# Autodesk Inventor assembly: ASY MSC 800 gills
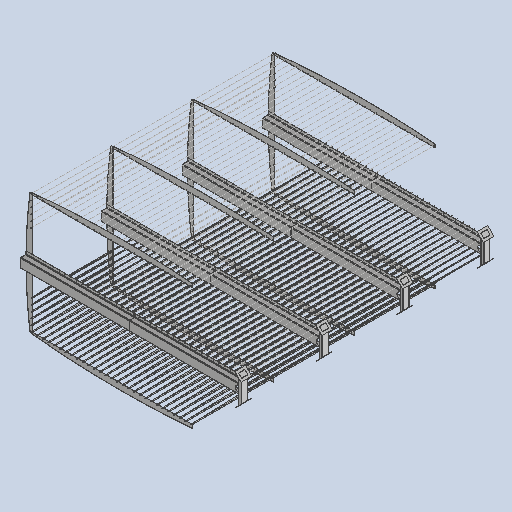
[picture p0: Inventor's stored thumbnail of the model, 512x512]
Saved by Autodesk Inventor 2025 (Build 290162010, 162A)
## iProperties
Created: 2024-08-31
Part Number: ASY MSC 800 gills
Document SubType Name: Assembly
Designer: pokla
Stock Number: ASY МОО 800 Жабры
Mass: 57918.9 g
Surface Area: 154099 cm^2
Volume: 7985.94 cm^3
Density: 7.25262 g/cm^3
Author: pokla
## Documents named in this file (14)
- C:\Users\DELL\YandexDisk-badmisterfox\домашниий пк\Inventor\Manturovo\Manturovo_Se-clar\ASY MSC 800 gills.iam
- C:\Users\DELL\YandexDisk-badmisterfox\домашниий пк\Inventor\Manturovo\Manturovo_Se-clar\MSC 804 sheet gills.ipt
- C:\Users\DELL\YandexDisk-badmisterfox\домашниий пк\Inventor\Manturovo\Manturovo_Se-clar\MSC 810 pillar gills.ipt
- C:\Users\DELL\YandexDisk-badmisterfox\домашниий пк\Inventor\Manturovo\Manturovo_Se-clar\MSC 805 sheet gills.ipt
- C:\Users\DELL\YandexDisk-badmisterfox\домашниий пк\Inventor\Manturovo\Manturovo_Se-clar\MSC 806 sheet gills.ipt
- C:\Users\DELL\YandexDisk-badmisterfox\домашниий пк\Inventor\Manturovo\Manturovo_Se-clar\MSC 807 sheet gills.ipt
- C:\Users\DELL\YandexDisk-badmisterfox\домашниий пк\Inventor\Manturovo\Manturovo_Se-clar\MSC 808 sheet gills.ipt
- C:\Users\DELL\YandexDisk-badmisterfox\домашниий пк\Inventor\Manturovo\Manturovo_Se-clar\MSC 809 sheet gills.ipt
- C:\Users\DELL\YandexDisk-badmisterfox\домашниий пк\Inventor\Manturovo\Manturovo_Se-clar\MSC 813 wall support gills.ipt
- C:\Users\DELL\YandexDisk-badmisterfox\домашниий пк\Inventor\Manturovo\Manturovo_Se-clar\MSC 811 pillar gills.ipt
- C:\Users\DELL\YandexDisk-badmisterfox\домашниий пк\Inventor\Manturovo\Manturovo_Se-clar\MSC 814 string for sheets gills.ipt
- C:\Users\DELL\YandexDisk-badmisterfox\домашниий пк\Inventor\Manturovo\Manturovo_Se-clar\MSC 812 top support gills.ipt
- C:\Users\DELL\YandexDisk-badmisterfox\домашниий пк\Inventor\Manturovo\Manturovo_Se-clar\MSC 803 sheet gills.ipt
- C:\Users\DELL\YandexDisk-badmisterfox\домашниий пк\Inventor\Manturovo\Manturovo_Se-clar\ASY MSC 800.1 gills base.iam
## Components (214 placed, 13 different names)
1. MSC 0203 sheet gills:1 — Angle:2, Tangent:8, Tangent:9, Flush:15, Flush:19
2. MSC 0204 sheet gills:1 — Angle:3, Tangent:10, Tangent:11, Flush:15, Flush:16
3. MSC 0205 sheet gills:1 — Angle:4, Tangent:12, Tangent:13, Flush:16, Flush:17
4. MSC 0206 sheet gills:1 — Angle:5, Tangent:17, Tangent:18, Flush:17, Flush:18
5. MSC 0207 sheet gills:1 — Angle:6, Tangent:19, Tangent:20, Flush:18
6. MSC 814 string for sheets gills:143 — Rigid:40
7. MSC 814 string for sheets gills:152 — Rigid:24
8. MSC 814 string for sheets gills:371
9. MSC 814 string for sheets gills:372
10. MSC 814 string for sheets gills:373
11. MSC 814 string for sheets gills:374
12. MSC 814 string for sheets gills:375
13. MSC 814 string for sheets gills:2 — Rigid:12
14. MSC 0201 sheet gills:1 — Rigid:33, Angle:2, Angle:3, Angle:4, Angle:5, Angle:6, Tangent:14, Tangent:15, Tangent:16, Flush:19
15. MSC 804 sheet gills:1 — Rigid:33
16. MSC 814 string for sheets gills:1 — Rotational:1
17. MSC 814 string for sheets gills:3 — Rotational:2
18. MSC 814 string for sheets gills:376 — Rotational:3
19. MSC 814 string for sheets gills:377
20. MSC 0201 sheet gills:2
21. MSC 804 sheet gills:2
22. MSC 814 string for sheets gills:378
23. MSC 814 string for sheets gills:379
24. MSC 814 string for sheets gills:380
25. MSC 814 string for sheets gills:381
26. MSC 0201 sheet gills:3
27. MSC 804 sheet gills:3
28. MSC 814 string for sheets gills:382
29. MSC 814 string for sheets gills:383
30. MSC 814 string for sheets gills:384
31. MSC 814 string for sheets gills:385
32. MSC 0201 sheet gills:4
33. MSC 804 sheet gills:4
34. MSC 814 string for sheets gills:386
35. MSC 814 string for sheets gills:387
36. MSC 814 string for sheets gills:388
37. MSC 814 string for sheets gills:389
38. MSC 0201 sheet gills:5
39. MSC 804 sheet gills:5
40. MSC 814 string for sheets gills:390
41. MSC 814 string for sheets gills:391
42. MSC 814 string for sheets gills:392
43. MSC 814 string for sheets gills:393
44. MSC 0201 sheet gills:6
45. MSC 804 sheet gills:6
46. MSC 814 string for sheets gills:394
47. MSC 814 string for sheets gills:395
48. MSC 814 string for sheets gills:396
49. MSC 814 string for sheets gills:397
50. MSC 0201 sheet gills:7
51. MSC 804 sheet gills:7
52. MSC 814 string for sheets gills:398
53. MSC 814 string for sheets gills:399
54. MSC 814 string for sheets gills:400
55. MSC 814 string for sheets gills:401
56. MSC 0201 sheet gills:8
57. MSC 804 sheet gills:8
58. MSC 814 string for sheets gills:402
59. MSC 814 string for sheets gills:403
60. MSC 814 string for sheets gills:404
61. MSC 814 string for sheets gills:405
62. MSC 0201 sheet gills:9
63. MSC 804 sheet gills:9
64. MSC 814 string for sheets gills:406
65. MSC 814 string for sheets gills:407
66. MSC 814 string for sheets gills:408
67. MSC 814 string for sheets gills:409
68. MSC 0201 sheet gills:10
69. MSC 804 sheet gills:10
70. MSC 814 string for sheets gills:410
71. MSC 814 string for sheets gills:411
72. MSC 814 string for sheets gills:412
73. MSC 814 string for sheets gills:413
74. MSC 0201 sheet gills:11
75. MSC 804 sheet gills:11
76. MSC 814 string for sheets gills:414
77. MSC 814 string for sheets gills:415
78. MSC 814 string for sheets gills:416
79. MSC 814 string for sheets gills:417
80. MSC 0201 sheet gills:12
81. MSC 804 sheet gills:12
82. MSC 814 string for sheets gills:418
83. MSC 814 string for sheets gills:419
84. MSC 814 string for sheets gills:420
85. MSC 814 string for sheets gills:421
86. MSC 0201 sheet gills:13
87. MSC 804 sheet gills:13
88. MSC 814 string for sheets gills:422
89. MSC 814 string for sheets gills:423
90. MSC 814 string for sheets gills:424
91. MSC 814 string for sheets gills:425
92. MSC 0201 sheet gills:14
93. MSC 804 sheet gills:14
94. MSC 814 string for sheets gills:426
95. MSC 814 string for sheets gills:427
96. MSC 814 string for sheets gills:428
97. MSC 814 string for sheets gills:429
98. MSC 0201 sheet gills:15
99. MSC 804 sheet gills:15
100. MSC 814 string for sheets gills:430
101. MSC 814 string for sheets gills:431
102. MSC 814 string for sheets gills:432
103. MSC 814 string for sheets gills:433
104. MSC 0201 sheet gills:16
105. MSC 804 sheet gills:16
106. MSC 814 string for sheets gills:434
107. MSC 814 string for sheets gills:435
108. MSC 814 string for sheets gills:436
109. MSC 814 string for sheets gills:437
110. MSC 0201 sheet gills:17
111. MSC 804 sheet gills:17
112. MSC 814 string for sheets gills:438
113. MSC 814 string for sheets gills:439
114. MSC 814 string for sheets gills:440
115. MSC 814 string for sheets gills:441
116. MSC 0201 sheet gills:18
117. MSC 804 sheet gills:18
118. MSC 814 string for sheets gills:442
119. MSC 814 string for sheets gills:443
120. MSC 814 string for sheets gills:444
121. MSC 814 string for sheets gills:445
122. MSC 0201 sheet gills:19
123. MSC 804 sheet gills:19
124. MSC 814 string for sheets gills:446
125. MSC 814 string for sheets gills:447
126. MSC 814 string for sheets gills:448
127. MSC 814 string for sheets gills:449
128. MSC 0201 sheet gills:20
129. MSC 804 sheet gills:20
130. MSC 814 string for sheets gills:450
131. MSC 814 string for sheets gills:451
132. MSC 814 string for sheets gills:452
133. MSC 814 string for sheets gills:453
134. MSC 0201 sheet gills:21
135. MSC 804 sheet gills:21
136. MSC 814 string for sheets gills:454
137. MSC 814 string for sheets gills:455
138. MSC 814 string for sheets gills:456
139. MSC 814 string for sheets gills:457
140. MSC 0201 sheet gills:22
141. MSC 804 sheet gills:22
142. MSC 814 string for sheets gills:458
143. MSC 814 string for sheets gills:459
144. MSC 814 string for sheets gills:460
145. MSC 814 string for sheets gills:461
146. MSC 0201 sheet gills:23
147. MSC 804 sheet gills:23
148. MSC 814 string for sheets gills:462
149. MSC 814 string for sheets gills:463
150. MSC 814 string for sheets gills:464
151. MSC 814 string for sheets gills:465
152. MSC 0201 sheet gills:24
153. MSC 804 sheet gills:24
154. MSC 814 string for sheets gills:466
155. MSC 814 string for sheets gills:467
156. MSC 814 string for sheets gills:468
157. MSC 814 string for sheets gills:469
158. MSC 0201 sheet gills:25
159. MSC 804 sheet gills:25
160. MSC 814 string for sheets gills:470
161. MSC 814 string for sheets gills:471
162. MSC 814 string for sheets gills:472
163. MSC 814 string for sheets gills:473
164. MSC 0201 sheet gills:26
165. MSC 804 sheet gills:26
166. MSC 814 string for sheets gills:474
167. MSC 814 string for sheets gills:475
168. MSC 814 string for sheets gills:476
169. MSC 814 string for sheets gills:477
170. MSC 0201 sheet gills:27
171. MSC 804 sheet gills:27
172. MSC 814 string for sheets gills:478
173. MSC 814 string for sheets gills:479
174. MSC 814 string for sheets gills:480
175. MSC 814 string for sheets gills:481
176. MSC 0201 sheet gills:28
177. MSC 804 sheet gills:28
178. MSC 814 string for sheets gills:482
179. MSC 814 string for sheets gills:483
180. MSC 814 string for sheets gills:484
181. MSC 814 string for sheets gills:485
182. MSC 0201 sheet gills:29
183. MSC 804 sheet gills:29
184. MSC 814 string for sheets gills:486
185. MSC 814 string for sheets gills:487
186. MSC 814 string for sheets gills:488
187. MSC 813 wall support gills:1 — Rigid:12, Rigid:30, Tangent:14, Tangent:15
188. MSC 812 top support gills:1 — Rigid:28, Rigid:30, Tangent:8, Tangent:9, Tangent:10, Tangent:11, Tangent:12, Tangent:13, Tangent:17, Tangent:18, Tangent:19, Tangent:20, Rigid:40
189. MSC 811 pillar gills:1 — Rigid:28, Rigid:29
190. MSC 812 top support gills:2 — Rigid:24, Rigid:29, Rigid:31
191. MSC 813 wall support gills:2 — Rigid:31, Rotational:3
192. MSC 810 pillar gills:1 — Rotational:1, Rotational:2, Tangent:16
193. ASY MSC 800.1 gills base:1 [sub-assembly]
194. MSC 813 wall support gills:4
195. MSC 812 top support gills:3
196. MSC 811 pillar gills:2
197. MSC 812 top support gills:4
198. MSC 813 wall support gills:5
199. MSC 810 pillar gills:2
200. ASY MSC 800.1 gills base:2 [sub-assembly]
201. MSC 813 wall support gills:6
202. MSC 812 top support gills:5
203. MSC 811 pillar gills:3
204. MSC 812 top support gills:6
205. MSC 813 wall support gills:7
206. MSC 810 pillar gills:3
207. ASY MSC 800.1 gills base:3 [sub-assembly]
208. MSC 813 wall support gills:8
209. MSC 812 top support gills:7
210. MSC 811 pillar gills:4
211. MSC 812 top support gills:8
212. MSC 813 wall support gills:9
213. MSC 810 pillar gills:4
214. ASY MSC 800.1 gills base:4 [sub-assembly]
## Component patterns: (6 elements, first: MSC 814 string for sheets gills:152), (29 elements, first: MSC 814 string for sheets gills:2 + MSC 0201 sheet gills:1 + MSC 804 sheet gills:1 + MSC 814 string for sheets gills:1 + MSC 814 string for sheets gills:3 + MSC 814 string for sheets gills:376), (4 elements, first: MSC 813 wall support gills:1 + MSC 812 top support gills:1 + MSC 811 pillar gills:1 + MSC 812 top support gills:2 + MSC 813 wall support gills:2 + MSC 810 pillar gills:1 + ASY MSC 800.1 gills base:1)
## Relationships (41: Tangent 13, WeldJoint 9, Flush 8, Angle 5, Mate 3, RevoluteJoint 3)
- [WeldJoint]: MSC 811 pillar gills:1 ↔ MSC 810 pillar gills:1
- [Flush]: MSC 810 pillar gills:1 ↔ ASY MSC 800.1 gills base:1
- [Mate]: MSC 810 pillar gills:1 ↔ ASY MSC 800.1 gills base:1
- [Flush] (5 mm): MSC 810 pillar gills:1 ↔ ASY MSC 800.1 gills base:1
- Rigid:12 [WeldJoint] (-5 mm): MSC 814 string for sheets gills:2 ↔ MSC 813 wall support gills:1
- [Mate]: ASY MSC 800.1 gills base:1
- [Mate]: ASY MSC 800.1 gills base:1
- [Flush]: ASY MSC 800.1 gills base:1
- Rigid:24 [WeldJoint] (-5 mm): MSC 814 string for sheets gills:152 ↔ MSC 812 top support gills:2
- Rigid:28 [WeldJoint]: MSC 812 top support gills:1 ↔ MSC 811 pillar gills:1
- Rigid:29 [WeldJoint]: MSC 811 pillar gills:1 ↔ MSC 812 top support gills:2
- Rigid:30 [WeldJoint]: MSC 813 wall support gills:1 ↔ MSC 812 top support gills:1
- Rigid:31 [WeldJoint]: MSC 812 top support gills:2 ↔ MSC 813 wall support gills:2
- Rotational:1 [RevoluteJoint] (5 mm): MSC 814 string for sheets gills:1 ↔ MSC 810 pillar gills:1
- Rotational:2 [RevoluteJoint] (-5 mm): MSC 814 string for sheets gills:3 ↔ MSC 810 pillar gills:1
- Rigid:33 [WeldJoint] (-10 mm): MSC 0201 sheet gills:1 ↔ MSC 804 sheet gills:1
- Angle:2 (0 deg): MSC 0203 sheet gills:1 ↔ MSC 0201 sheet gills:1
- Angle:3 (0 deg): MSC 0204 sheet gills:1 ↔ MSC 0201 sheet gills:1
- Angle:4 (0 deg): MSC 0205 sheet gills:1 ↔ MSC 0201 sheet gills:1
- Angle:5 (0 deg): MSC 0206 sheet gills:1 ↔ MSC 0201 sheet gills:1
- Angle:6 (0 deg): MSC 0207 sheet gills:1 ↔ MSC 0201 sheet gills:1
- Tangent:8: MSC 0203 sheet gills:1 ↔ MSC 812 top support gills:1
- Tangent:9: MSC 0203 sheet gills:1 ↔ MSC 812 top support gills:1
- Tangent:10: MSC 0204 sheet gills:1 ↔ MSC 812 top support gills:1
- Tangent:11: MSC 0204 sheet gills:1 ↔ MSC 812 top support gills:1
- Tangent:12: MSC 0205 sheet gills:1 ↔ MSC 812 top support gills:1
- Tangent:13: MSC 0205 sheet gills:1 ↔ MSC 812 top support gills:1
- Tangent:14: MSC 0201 sheet gills:1 ↔ MSC 813 wall support gills:1
- Tangent:15: MSC 0201 sheet gills:1 ↔ MSC 813 wall support gills:1
- Tangent:16: MSC 0201 sheet gills:1 ↔ MSC 810 pillar gills:1
- Tangent:17: MSC 0206 sheet gills:1 ↔ MSC 812 top support gills:1
- Tangent:18: MSC 0206 sheet gills:1 ↔ MSC 812 top support gills:1
- Tangent:19: MSC 0207 sheet gills:1 ↔ MSC 812 top support gills:1
- Tangent:20: MSC 0207 sheet gills:1 ↔ MSC 812 top support gills:1
- Flush:15: MSC 0203 sheet gills:1 ↔ MSC 0204 sheet gills:1
- Flush:16: MSC 0204 sheet gills:1 ↔ MSC 0205 sheet gills:1
- Flush:17: MSC 0205 sheet gills:1 ↔ MSC 0206 sheet gills:1
- Flush:18: MSC 0206 sheet gills:1 ↔ MSC 0207 sheet gills:1
- Flush:19: MSC 0203 sheet gills:1 ↔ MSC 0201 sheet gills:1
- Rigid:40 [WeldJoint] (5 mm): MSC 814 string for sheets gills:143 ↔ MSC 812 top support gills:1
- Rotational:3 [RevoluteJoint] (-5 mm): MSC 814 string for sheets gills:376 ↔ MSC 813 wall support gills:2
